# Autodesk Inventor assembly: bikeLockMountV2Assem
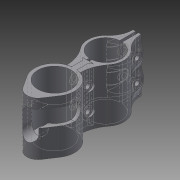
[picture p0: Inventor's stored thumbnail of the model, 180x180]
Saved by Autodesk Inventor 2015 (Build 190159000, 159)
## iProperties
Created: 2015-01-18
Part Number: bikeLockMountV2Assem
Document SubType Name: Assembly
Designer: rmsin_000
Author: rmsin_000
## Documents named in this file (3)
- C:\Users\rmsin_000\Desktop\MAKEiT\CAD\bikeLockMountV2Assem.iam
- C:\Users\rmsin_000\Desktop\MAKEiT\CAD\bikeLockMountV2part1.ipt
- C:\Users\rmsin_000\Desktop\MAKEiT\CAD\bikeLockMountV2part2.ipt
## Components (2 placed, 2 different names)
1. bikeLockMountV2part1:1 — Mate:1, Mate:2, Mate:3
2. bikeLockMountV2part2:1 — Mate:1, Mate:2, Mate:3
## Relationships (3: Mate 3)
- Mate:1: bikeLockMountV2part1:1 ↔ bikeLockMountV2part2:1
- Mate:2: bikeLockMountV2part1:1 ↔ bikeLockMountV2part2:1
- Mate:3: bikeLockMountV2part1:1 ↔ bikeLockMountV2part2:1
